# Autodesk Inventor assembly: Assembly_Opentrons_Autofocus_v3
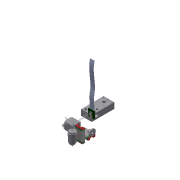
[picture p0: Inventor's stored thumbnail of the model, 180x180]
Saved by Autodesk Inventor 2019.4 (Build 234330000, 330)
## iProperties
Created: 2020-10-23
Part Number: Assembly_Opentrons_Autofocus_v3
Document SubType Name: Assembly
Designer: diederichbenedict
Author: diederichbenedict
## Documents named in this file (11)
- C:\Users\diederichbenedict\Dropbox\Dokumente\Promotion\PROJECTS\OPENTRONS\INVENTOR\Assembly_Opentrons_Autofocus_v3.iam
- C:\Users\diederichbenedict\Dropbox\Dokumente\Promotion\PROJECTS\OPENTRONS\INVENTOR\00_RasPi_Camera.ipt
- C:\Users\diederichbenedict\Dropbox\Dokumente\Promotion\PROJECTS\OPENTRONS\INVENTOR\00_spindel_slide.ipt
- C:\Users\diederichbenedict\Dropbox\Dokumente\Promotion\PROJECTS\OPENTRONS\INVENTOR\00_opticalpath.ipt
- C:\Users\diederichbenedict\Dropbox\Dokumente\Promotion\PROJECTS\OPENTRONS\INVENTOR\00_COMAR_Mirror_10mm.ipt
- C:\Users\diederichbenedict\Dropbox\Dokumente\Promotion\PROJECTS\OPENTRONS\INVENTOR\00_NEMA11.iam
- C:\Users\diederichbenedict\Dropbox\Dokumente\Promotion\PROJECTS\OPENTRONS\INVENTOR\00_objectivelens_10x.ipt
- C:\Users\diederichbenedict\Dropbox\Dokumente\Promotion\PROJECTS\OPENTRONS\INVENTOR\01_Slide_camera_v1.ipt
- C:\Users\diederichbenedict\Dropbox\Dokumente\Promotion\PROJECTS\OPENTRONS\INVENTOR\00_MGN12H, LINEAR GUIDE BLOCK.ipt
- C:\Users\diederichbenedict\Dropbox\Dokumente\Promotion\PROJECTS\OPENTRONS\INVENTOR\STL\00_gear_rack.ipt
- C:\Users\diederichbenedict\Dropbox\Dokumente\Promotion\PROJECTS\OPENTRONS\INVENTOR\STL\00_gear_nema.ipt
## Components (11 placed, 10 different names)
1. 00_opticalpath:1 — Insert:9, Insert:11, Insert:12
2. 00_COMAR_Mirror_10mm:1 — Insert:11
3. 00_RasPi_Camera:1 — Insert:12, Angle:2
4. 00_MGN12H, LINEAR GUIDE BLOCK:1 — Mate:2, Angle:3, Flush:5, Flush:6, Angle:4, Mate:5
5. 00_spindel_slide:1
6. 00_NEMA11:2 [sub-assembly] — Flush:6, Angle:4, Mate:3, Mate:5, Mate:6
7. 00_objectivelens_10x:1 — Insert:9, Flush:7, Tangent:1
8. 00_gear_rack:1 — Mate:4, Angle:5, Flush:8, Mate:7
9. 00_gear_nema:1 — Mate:3
10. 00_MGN12H, LINEAR GUIDE BLOCK:2 — Mate:2, Angle:3, Flush:5, Mate:4, Angle:5, Flush:7, Flush:8, Mate:6, Mate:7, Tangent:1
11. 01_Slide_camera_v1:1
## Relationships (19: Mate 6, Flush 5, Angle 4, Insert 3, Tangent 1)
- [Flush]: 00_MGN12H, LINEAR GUIDE BLOCK:1 ↔ 00_objectivelens_10x:1
- Insert:9: 00_opticalpath:1 ↔ 00_objectivelens_10x:1
- Insert:11: 00_opticalpath:1 ↔ 00_COMAR_Mirror_10mm:1
- Insert:12: 00_opticalpath:1 ↔ 00_RasPi_Camera:1
- Angle:2 (0 deg): 00_RasPi_Camera:1
- Mate:2 (10 mm): 00_MGN12H, LINEAR GUIDE BLOCK:1 ↔ 00_MGN12H, LINEAR GUIDE BLOCK:2
- Angle:3 (0 deg): 00_MGN12H, LINEAR GUIDE BLOCK:1 ↔ 00_MGN12H, LINEAR GUIDE BLOCK:2
- Flush:5: 00_MGN12H, LINEAR GUIDE BLOCK:1 ↔ 00_MGN12H, LINEAR GUIDE BLOCK:2
- Flush:6 (1 mm): 00_MGN12H, LINEAR GUIDE BLOCK:1 ↔ 00_NEMA11:2
- Angle:4 (0 deg): 00_MGN12H, LINEAR GUIDE BLOCK:1 ↔ 00_NEMA11:2
- Mate:3: 00_NEMA11:2 ↔ 00_gear_nema:1
- Mate:4 (-5 mm): 00_gear_rack:1 ↔ 00_MGN12H, LINEAR GUIDE BLOCK:2
- Angle:5 (0 deg): 00_gear_rack:1 ↔ 00_MGN12H, LINEAR GUIDE BLOCK:2
- Flush:7 (-8 mm): 00_objectivelens_10x:1 ↔ 00_MGN12H, LINEAR GUIDE BLOCK:2
- Flush:8: 00_gear_rack:1 ↔ 00_MGN12H, LINEAR GUIDE BLOCK:2
- Mate:5 (2 mm): 00_MGN12H, LINEAR GUIDE BLOCK:1 ↔ 00_NEMA11:2
- Mate:6 (7 mm): 00_NEMA11:2 ↔ 00_MGN12H, LINEAR GUIDE BLOCK:2
- Mate:7: 00_gear_rack:1 ↔ 00_MGN12H, LINEAR GUIDE BLOCK:2
- Tangent:1 (2 mm): 00_objectivelens_10x:1 ↔ 00_MGN12H, LINEAR GUIDE BLOCK:2
